# Autodesk Inventor assembly: LiftPrototypeMKI
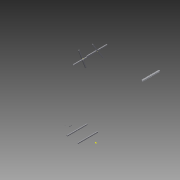
[picture p0: Inventor's stored thumbnail of the model, 180x180]
Saved by Autodesk Inventor 2013 (Build 170138000, 138)
## iProperties
Created: 2013-10-02
Part Number: LiftPrototypeMKI
Document SubType Name: Assembly
Designer: cobrooks
Author: cobrooks
## Documents named in this file (6)
- C:\Users\cobrooks\Documents\Robotics\2013-14\CAD\Lift\LiftPrototype\LiftPrototypeMKI.iam
- \\lmss\STUDENTS\Robotics\CAD Files\COTS Parts\Bosch Extrusion\Bosch 20x20.ipt
- \\lmss\STUDENTS\Robotics\CAD Files\5x5mm Box Aluminum.ipt
- \\lmss\STUDENTS\Robotics\CAD Files\COTS Parts\Fasteners\14-20 Washer - Flat.ipt
- \\lmss\STUDENTS\Robotics\CAD Files\COTS Parts\Fasteners\8-32 BHCS x1500.ipt
- \\lmss\STUDENTS\Robotics\CAD Files\COTS Parts\Fasteners\8-32 locknut.ipt
## Components (16 placed, 5 different names)
1. Bosch 20x20:1
2. 14-20 Washer - Flat:1 — Insert:2, Insert:3
3. 5x5mm Box Aluminum:1 — Insert:1, Insert:2
4. 5x5mm Box Aluminum:2 — Insert:3, Insert:4
5. 8-32 BHCS x1500:1 — Insert:1
6. 8-32 locknut:1 — Insert:4
7. 5x5mm Box Aluminum:3 — Insert:5, Insert:6
8. 5x5mm Box Aluminum:4 — Insert:7, Insert:8
9. 8-32 BHCS x1500:2 — Insert:5
10. 8-32 locknut:2 — Insert:8
11. 14-20 Washer - Flat:3 — Insert:6, Insert:7
12. 14-20 Washer - Flat:4
13. 5x5mm Box Aluminum:5
14. 5x5mm Box Aluminum:6
15. 8-32 BHCS x1500:3
16. 8-32 locknut:3
## Relationships (8: Insert 8)
- Insert:1: 5x5mm Box Aluminum:1 ↔ 8-32 BHCS x1500:1
- Insert:2: 14-20 Washer - Flat:1 ↔ 5x5mm Box Aluminum:1
- Insert:3: 14-20 Washer - Flat:1 ↔ 5x5mm Box Aluminum:2
- Insert:4: 5x5mm Box Aluminum:2 ↔ 8-32 locknut:1
- Insert:5: 5x5mm Box Aluminum:3 ↔ 8-32 BHCS x1500:2
- Insert:6: 5x5mm Box Aluminum:3 ↔ 14-20 Washer - Flat:3
- Insert:7: 5x5mm Box Aluminum:4 ↔ 14-20 Washer - Flat:3
- Insert:8: 5x5mm Box Aluminum:4 ↔ 8-32 locknut:2
